# Autodesk Inventor assembly: launcher.mainAssembly2
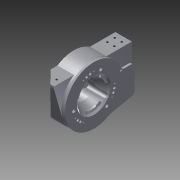
[picture p0: Inventor's stored thumbnail of the model, 180x180]
Saved by Autodesk Inventor 2011 (Build 150239000, 239)
## iProperties
Created: 2011-04-12
Part Number: launcher.mainAssembly2
Document SubType Name: Assembly
Designer: Rob
Author: Rob
## Documents named in this file (6)
- C:\Users\M. Woods III\Desktop\design\Mechanical Drawings\launcher_2.iam
- C:\Users\M. Woods III\Desktop\design\Mechanical Drawings\launcher_2_housing.ipt
- C:\Users\M. Woods III\Desktop\design\Mechanical Drawings\launcher_3x8x4_bearing.ipt
- C:\Users\M. Woods III\Desktop\design\Mechanical Drawings\launcher_latch.ipt
- C:\Users\M. Woods III\Desktop\design\Mechanical Drawings\launcher_cam.ipt
- C:\Users\M. Woods III\Desktop\design\Mechanical Drawings\launcher_2_cap.ipt
## Components (12 placed, 5 different names)
1. launcher_2_housing:1 — Mate:1, Mate:2, Mate:3, Mate:4, Mate:5, Mate:6, Mate:7, Mate:8, Mate:9, Mate:10, Mate:11, Mate:12, Mate:13, Mate:14, Mate:15, Mate:16, Mate:18
2. launcher_3x8x4_bearing:1 — Mate:3, Mate:4
3. launcher_3x8x4_bearing:2 — Mate:5, Mate:6
4. launcher_3x8x4_bearing:3 — Mate:1, Mate:2
5. launcher_3x8x4_bearing:4 — Mate:7, Mate:8
6. launcher_3x8x4_bearing:5 — Mate:11, Mate:12
7. launcher_3x8x4_bearing:6 — Mate:9, Mate:10
8. launcher_cam:1 — Mate:15, Mate:16, Mate:17
9. launcher_2_cap:1 — Mate:17, Mate:18, Mate:19
10. launcher_latch:1 — Mate:13, Mate:14
11. launcher_latch:2 — Mate:19
12. launcher_latch:3
## Component patterns: (3 elements, first: launcher_latch:1)
## Relationships (19: Mate 19)
- Mate:1: launcher_2_housing:1 ↔ launcher_3x8x4_bearing:3
- Mate:2: launcher_2_housing:1 ↔ launcher_3x8x4_bearing:3
- Mate:3: launcher_2_housing:1 ↔ launcher_3x8x4_bearing:1
- Mate:4: launcher_2_housing:1 ↔ launcher_3x8x4_bearing:1
- Mate:5: launcher_2_housing:1 ↔ launcher_3x8x4_bearing:2
- Mate:6: launcher_2_housing:1 ↔ launcher_3x8x4_bearing:2
- Mate:7: launcher_2_housing:1 ↔ launcher_3x8x4_bearing:4
- Mate:8: launcher_2_housing:1 ↔ launcher_3x8x4_bearing:4
- Mate:9: launcher_2_housing:1 ↔ launcher_3x8x4_bearing:6
- Mate:10: launcher_2_housing:1 ↔ launcher_3x8x4_bearing:6
- Mate:11: launcher_2_housing:1 ↔ launcher_3x8x4_bearing:5
- Mate:12: launcher_2_housing:1 ↔ launcher_3x8x4_bearing:5
- Mate:13: launcher_2_housing:1 ↔ launcher_latch:1
- Mate:14: launcher_2_housing:1 ↔ launcher_latch:1
- Mate:15: launcher_2_housing:1 ↔ launcher_cam:1
- Mate:16: launcher_2_housing:1 ↔ launcher_cam:1
- Mate:17: launcher_cam:1 ↔ launcher_2_cap:1
- Mate:18: launcher_2_housing:1 ↔ launcher_2_cap:1
- Mate:19: launcher_2_cap:1 ↔ launcher_latch:2
